# Autodesk Inventor assembly: 2f1
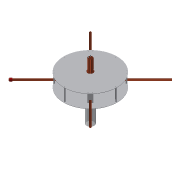
[picture p0: Inventor's stored thumbnail of the model, 180x180]
Saved by Autodesk Inventor 2017 (Build 210142000, 142)
## iProperties
Created: 2013-05-22
Part Number: 2f1
Document SubType Name: Assembly
Designer: Dave
Description: Feed dipole
Author: Dave
## Documents named in this file (12)
- C:\Users\krosie\Google Drive\HERA\hera-cad\feed\dipole.iam
- C:\Users\krosie\Google Drive\HERA\hera-cad\feed\dipoleBottomDisc.ipt
- C:\Users\krosie\Google Drive\HERA\hera-cad\feed\dipoleArm.ipt
- C:\Users\krosie\Google Drive\HERA\hera-cad\feed\dipoleDiscSpacer.ipt
- C:\Users\krosie\Google Drive\HERA\hera-cad\feed\dipoleMast.ipt
- C:\Users\krosie\Google Drive\HERA\hera-cad\feed\dipoleArmHold.ipt
- C:\Users\krosie\Google Drive\HERA\hera-cad\feed\dipoleArmRest.ipt
- C:\Users\krosie\Google Drive\HERA\hera-cad\feed\dipoleTopDisc.ipt
- C:\Users\krosie\Google Drive\HERA\hera-cad\feed\matingBoard.ipt
- C:\Users\krosie\Google Drive\HERA\hera-cad\feed\roundNorthBand.ipt
- C:\Users\krosie\Google Drive\HERA\hera-cad\feed\balun.ipt
- C:\Users\krosie\Google Drive\HERA\hera-cad\feed\collar_paper.ipt
## Components (23 placed, 11 different names)
1. dipoleBottomDisc:1 — Insert:5, Insert:8, Insert:9, Insert:12, Insert:13, Insert:18, Insert:19, Insert:20
2. dipoleDiscSpacer:2 — Insert:5, Insert:21
3. dipoleDiscSpacer:3 — Insert:18, Insert:22
4. dipoleDiscSpacer:4 — Insert:19
5. dipoleDiscSpacer:5 — Insert:20
6. dipoleTopDisc:1 — Insert:21, Insert:22, Insert:23, Mate:2
7. matingBoard:1 — Insert:10, Insert:11, Insert:12, Insert:13, Insert:27
8. collar_paper:1 — Mate:1, Mate:2, Angle:1
9. dipoleMast:1 — Insert:23, Mate:1
10. roundNorthBand:1 — Insert:26, Angle:1
11. balun:1 — Insert:27
12. dipoleArmHold:1 — Insert:4, Insert:8, Insert:9
13. dipoleArm:1 — Insert:4, Insert:26
14. dipoleArmRest:1 — Insert:10, Insert:11
15. dipoleArmHold:2
16. dipoleArm:2
17. dipoleArmRest:2
18. dipoleArmHold:3
19. dipoleArm:3
20. dipoleArmRest:3
21. dipoleArmHold:4
22. dipoleArm:4
23. dipoleArmRest:4
## Component patterns: arms (4 elements)
## Relationships (19: Insert 16, Mate 2, Angle 1)
- Insert:4 (-275.59 mm): dipoleArmHold:1 ↔ dipoleArm:1
- Insert:5: dipoleBottomDisc:1 ↔ dipoleDiscSpacer:2
- Insert:8: dipoleBottomDisc:1 ↔ dipoleArmHold:1
- Insert:9: dipoleBottomDisc:1 ↔ dipoleArmHold:1
- Insert:10: matingBoard:1 ↔ dipoleArmRest:1
- Insert:11: matingBoard:1 ↔ dipoleArmRest:1
- Insert:12: dipoleBottomDisc:1 ↔ matingBoard:1
- Insert:13: dipoleBottomDisc:1 ↔ matingBoard:1
- Insert:18: dipoleBottomDisc:1 ↔ dipoleDiscSpacer:3
- Insert:19: dipoleBottomDisc:1 ↔ dipoleDiscSpacer:4
- Insert:20: dipoleBottomDisc:1 ↔ dipoleDiscSpacer:5
- Insert:21: dipoleDiscSpacer:2 ↔ dipoleTopDisc:1
- Insert:22: dipoleDiscSpacer:3 ↔ dipoleTopDisc:1
- Insert:23: dipoleTopDisc:1 ↔ dipoleMast:1
- Insert:26 (-30 mm): roundNorthBand:1 ↔ dipoleArm:1
- Insert:27: matingBoard:1 ↔ balun:1
- Mate:1: collar_paper:1 ↔ dipoleMast:1
- Mate:2: dipoleTopDisc:1 ↔ collar_paper:1
- Angle:1 (0 deg): collar_paper:1 ↔ roundNorthBand:1
